# Autodesk Inventor assembly: template
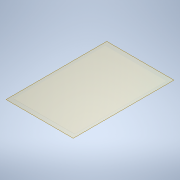
[picture p0: Inventor's stored thumbnail of the model, 180x180]
Saved by Autodesk Inventor 2020 (Build 240168000, 168)
## iProperties
Created: 2021-08-27
Part Number: template
Document SubType Name: Assembly
Designer: Masato
Author: Masato
## Documents named in this file (2)
- C:\Users\Masato\Documents\Inventor\CIT Brains_Inventor\OpenPlatform_ver3_0\cam\template.iam
- C:\Users\Masato\Documents\Inventor\CIT Brains_Inventor\OpenPlatform_ver3_0\cam\Disposable_Board.ipt
## Components (1 placed, 1 different names)
1. Disposable_Board:1 — メイト:2, メイト:1, フラッシュ:1, フラッシュ:2
## Relationships (4: Mate 2, Flush 2)
- メイト:2 [Mate]: Disposable_Board:1
- メイト:1 [Mate]: Disposable_Board:1
- フラッシュ:1 [Flush]: Disposable_Board:1
- フラッシュ:2 [Flush]: Disposable_Board:1
